# Autodesk Inventor assembly: High Strength 36-tooth Gear-Free Spinning Insert
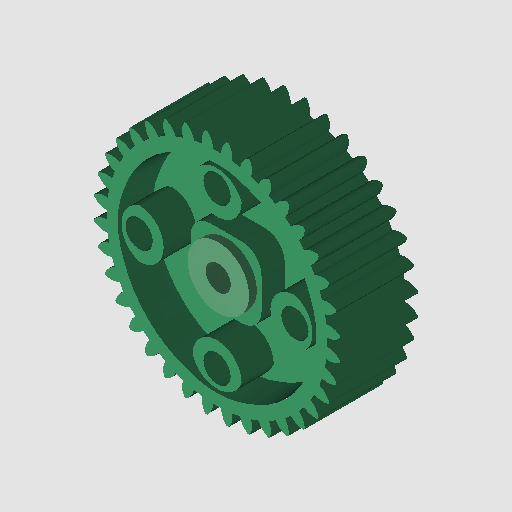
[picture p0: Inventor's stored thumbnail of the model, 512x512]
Saved by Autodesk Inventor 2018 (Build 220112000, 112)
## iProperties
Category: Motion
Company: Super Sonic Sparks, Team 24
Document SubType Name: Assembly
Designer: Jordan Kiesel
Catalog Web Link: http://www.vexrobotics.com/products/accessories/motion/276-2250.html
Description: High strength free spinning idler gear.
Vendor: VEX Robotics, Inc.
Created: 2017-12-12
Author: Jordan Kiesel
Title: High Strength 36-tooth Gear-Free Spinning Insert
Comments: Build mechanisms capable of withstanding higher stresses than ever before. Lift heavier loads, and survive bigger impacts with high strength gears. ▷ High strength gears mate with all VEX spur gears. ▷ Double-thick face width provides added tooth strength. ▷ Use the round-hole inserts to build free spinning idler gears. ▷ Build gearboxes that resist high shock-loads. ▷ Bolt Gears together for added strength.
## Documents named in this file (3)
- D:\Google Drive\5776E 17'-18'\ßid's Stuff\CAD Location 17'-18'\Inventor\Vex In The Zone\Resources\2016 BNS CAD Library (beta)\Motion\Spur Gears\High Strength 36-tooth Gear-Free Spinning Insert.iam
- D:\Google Drive\5776E 17'-18'\ßid's Stuff\CAD Location 17'-18'\Inventor\Vex In The Zone\Resources\2016 BNS CAD Library (beta)\Motion\Spur Gears\Reference Parts\High Strength Gears\High Strength 36-tooth Gear.ipt
- D:\Google Drive\5776E 17'-18'\ßid's Stuff\CAD Location 17'-18'\Inventor\Vex In The Zone\Resources\2016 BNS CAD Library (beta)\Motion\Reference Parts\Free Spinning Gear Insert.ipt
## Components (3 placed, 2 different names)
1. High Strength 36-tooth Gear:1 — Mate:1, Mate:2, Mate:3, Mate:4, Mate:5, Mate:6
2. Free Spinning Gear Insert:1 — Mate:1, Mate:2, Mate:3
3. Free Spinning Gear Insert:2 — Mate:4, Mate:5, Mate:6
## Relationships (6: Mate 6)
- Mate:1: High Strength 36-tooth Gear:1 ↔ Free Spinning Gear Insert:1
- Mate:2 (0.0254 mm): High Strength 36-tooth Gear:1 ↔ Free Spinning Gear Insert:1
- Mate:3 (0.0254 mm): High Strength 36-tooth Gear:1 ↔ Free Spinning Gear Insert:1
- Mate:4: High Strength 36-tooth Gear:1 ↔ Free Spinning Gear Insert:2
- Mate:5 (0.0254 mm): High Strength 36-tooth Gear:1 ↔ Free Spinning Gear Insert:2
- Mate:6 (0.0254 mm): High Strength 36-tooth Gear:1 ↔ Free Spinning Gear Insert:2
